# Autodesk Inventor assembly: Assembly2
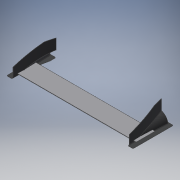
[picture p0: Inventor's stored thumbnail of the model, 180x180]
Saved by Autodesk Inventor 2018.1 (Build 221171000, 171)
## iProperties
Created: 2017-11-02
Part Number: Assembly2
Material: 一般
Document SubType Name: Assembly
Designer: kuwano
Author: kuwano
## Documents named in this file (4)
- D:\kuwano\Documents\Inventor\KITformula\AeroCAD2018\CAD\Inventor\Aero Parts\F-wing\test\Assembly2.iam
- D:\kuwano\Documents\Inventor\KITformula\AeroCAD2018\CAD\Inventor\Aero Parts\F-wing\test\test_front_end_plate.ipt
- D:\kuwano\Documents\Inventor\KITformula\AeroCAD2018\CAD\Inventor\Aero Parts\F-wing\test\test_front_end_plate_MIR.ipt
- D:\kuwano\Documents\Inventor\KITformula\AeroCAD2018\CAD\Inventor\Aero Parts\F-wing\test\test_base.ipt
## Components (3 placed, 3 different names)
1. test_front_end_plate:1 — フラッシュ:1, フラッシュ:2, メイト:3, メイト:4
2. test_front_end_plate_MIR:1 — フラッシュ:1, フラッシュ:2
3. test_base:1 — メイト:5
## Relationships (5: Mate 3, Flush 2)
- フラッシュ:1 [Flush]: test_front_end_plate:1 ↔ test_front_end_plate_MIR:1
- フラッシュ:2 [Flush]: test_front_end_plate:1 ↔ test_front_end_plate_MIR:1
- メイト:3 [Mate] (580 mm): test_front_end_plate:1
- メイト:4 [Mate]: test_front_end_plate:1
- メイト:5 [Mate]: test_base:1
